# Autodesk Inventor assembly: Electrical Feedthrough Collar
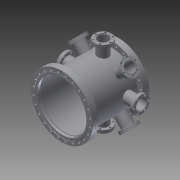
[picture p0: Inventor's stored thumbnail of the model, 180x180]
Saved by Autodesk Inventor 2015 (Build 190159000, 159)
## iProperties
Created: 2014-05-19
Part Number: Electrical Feedthrough Collar
Document SubType Name: Assembly
Designer: ijs09
Author: ijs09
## Documents named in this file (4)
- D:\Inventor\CCM CAD Files\CADFiles\EDM Machine\Electrical and Microwave Feedthrough Collar\Electrical Feedthrough Collar.iam
- D:\Inventor\CCM CAD Files\CADFiles\EDM Machine\Electrical and Microwave Feedthrough Collar\Vacuum Cylinder.ipt
- D:\Inventor\CCM CAD Files\CADFiles\EDM Machine\Electrical and Microwave Feedthrough Collar\DN200CF.ipt
- D:\Inventor\CCM CAD Files\CADFiles\EDM Machine\Electrical and Microwave Feedthrough Collar\DN35CF Counter Bored.ipt
## Components (11 placed, 3 different names)
1. Vacuum Cylinder:1 — Mate:1, Mate:2, Mate:3, Mate:4, Mate:5, Mate:6, Mate:7, Mate:8, Mate:9, Mate:10, Mate:13, Mate:14, Mate:15, Mate:16, Mate:18, Mate:19, Mate:20, Mate:21, Mate:22, Mate:23
2. DN200CF:1 — Mate:3, Mate:4, Mate:17
3. DN200CF:2 — Mate:1, Mate:2, Mate:17
4. DN35CF Counter Bored:1 — Mate:9, Mate:10, Symmetry:1
5. DN35CF Counter Bored:2 — Mate:7, Mate:8
6. DN35CF Counter Bored:3 — Mate:5, Mate:6, Symmetry:1
7. DN35CF Counter Bored:4 — Mate:15, Mate:16
8. DN35CF Counter Bored:5 — Mate:13, Mate:14
9. DN35CF Counter Bored:6 — Mate:18, Mate:19
10. DN35CF Counter Bored:7 — Mate:20, Mate:21
11. DN35CF Counter Bored:8 — Mate:22, Mate:23
## Relationships (22: Mate 21, Symmetry 1)
- Mate:1: Vacuum Cylinder:1 ↔ DN200CF:2
- Mate:2: Vacuum Cylinder:1 ↔ DN200CF:2
- Mate:3: Vacuum Cylinder:1 ↔ DN200CF:1
- Mate:4: Vacuum Cylinder:1 ↔ DN200CF:1
- Mate:5: Vacuum Cylinder:1 ↔ DN35CF Counter Bored:3
- Mate:6: Vacuum Cylinder:1 ↔ DN35CF Counter Bored:3
- Mate:7: Vacuum Cylinder:1 ↔ DN35CF Counter Bored:2
- Mate:8: Vacuum Cylinder:1 ↔ DN35CF Counter Bored:2
- Mate:9: Vacuum Cylinder:1 ↔ DN35CF Counter Bored:1
- Mate:10: Vacuum Cylinder:1 ↔ DN35CF Counter Bored:1
- Mate:13: Vacuum Cylinder:1 ↔ DN35CF Counter Bored:5
- Mate:14: Vacuum Cylinder:1 ↔ DN35CF Counter Bored:5
- Mate:15: Vacuum Cylinder:1 ↔ DN35CF Counter Bored:4
- Mate:16: Vacuum Cylinder:1 ↔ DN35CF Counter Bored:4
- Mate:17: DN200CF:1 ↔ DN200CF:2
- Symmetry:1: DN35CF Counter Bored:1 ↔ DN35CF Counter Bored:3
- Mate:18: Vacuum Cylinder:1 ↔ DN35CF Counter Bored:6
- Mate:19: Vacuum Cylinder:1 ↔ DN35CF Counter Bored:6
- Mate:20: Vacuum Cylinder:1 ↔ DN35CF Counter Bored:7
- Mate:21: Vacuum Cylinder:1 ↔ DN35CF Counter Bored:7
- Mate:22: Vacuum Cylinder:1 ↔ DN35CF Counter Bored:8
- Mate:23: Vacuum Cylinder:1 ↔ DN35CF Counter Bored:8
